# Autodesk Inventor assembly: Clamp with Piston Assembly
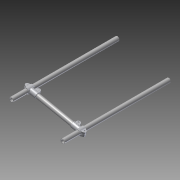
[picture p0: Inventor's stored thumbnail of the model, 180x180]
Saved by Autodesk Inventor 2014 (Build 180170000, 170)
## iProperties
Created: 2014-01-12
Part Number: Clamp with Piston Assembly
Document SubType Name: Assembly
Designer: Michael
Mass: 1489.5 g
Surface Area: 1855.4 cm^2
Volume: 236.743 cm^3
Density: 6.29163 g/cm^3
Author: Michael
## Documents named in this file (4)
- C:\Users\Michael\Documents\GitHub\2014buildCAD\Collector\Clamp with Piston Assembly.iam
- C:\Users\Michael\Documents\GitHub\2014buildCAD\Collector\Metal Pipe Connector 2 (9578T170).ipt
- C:\Users\Michael\Documents\GitHub\2014buildCAD\Collector\Steel Pipe 1-2 in (4347K311).ipt
- C:\Users\Michael\Documents\GitHub\2014buildCAD\Collector\Steel Pipe (Middle) 1-2 in (4347K311).ipt
## Components (5 placed, 3 different names)
1. Metal Pipe Connector 2 (9578T170):1 — Mate:1, Flush:1, Mate:5, Mate:6
2. Metal Pipe Connector 2 (9578T170):2 — Mate:2, Flush:2, Mate:3, Mate:4
3. Steel Pipe 1-2 in (4347K311):1 — Mate:1, Flush:1, Angle:1, Mate:7, Angle:2
4. Steel Pipe 1-2 in (4347K311):2 — Mate:2, Flush:2, Angle:1, Mate:7
5. Steel Pipe (Middle) 1-2 in (4347K311):1 — Mate:3, Mate:4, Mate:5, Mate:6, Angle:2
## Relationships (11: Mate 7, Flush 2, Angle 2)
- Mate:1: Metal Pipe Connector 2 (9578T170):1 ↔ Steel Pipe 1-2 in (4347K311):1
- Flush:1 (76.2 mm): Metal Pipe Connector 2 (9578T170):1 ↔ Steel Pipe 1-2 in (4347K311):1
- Mate:2: Metal Pipe Connector 2 (9578T170):2 ↔ Steel Pipe 1-2 in (4347K311):2
- Flush:2 (76.2 mm): Metal Pipe Connector 2 (9578T170):2 ↔ Steel Pipe 1-2 in (4347K311):2
- Mate:3: Metal Pipe Connector 2 (9578T170):2 ↔ Steel Pipe (Middle) 1-2 in (4347K311):1
- Mate:4 (-25.4 mm): Metal Pipe Connector 2 (9578T170):2 ↔ Steel Pipe (Middle) 1-2 in (4347K311):1
- Mate:5: Metal Pipe Connector 2 (9578T170):1 ↔ Steel Pipe (Middle) 1-2 in (4347K311):1
- Mate:6 (-25.4 mm): Metal Pipe Connector 2 (9578T170):1 ↔ Steel Pipe (Middle) 1-2 in (4347K311):1
- Angle:1 (0 deg): Steel Pipe 1-2 in (4347K311):1 ↔ Steel Pipe 1-2 in (4347K311):2
- Mate:7: Steel Pipe 1-2 in (4347K311):1 ↔ Steel Pipe 1-2 in (4347K311):2
- Angle:2 (0 deg): Steel Pipe 1-2 in (4347K311):1 ↔ Steel Pipe (Middle) 1-2 in (4347K311):1
